# Autodesk Inventor assembly: ReleaseAssembly
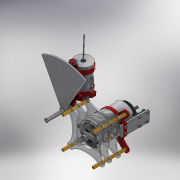
[picture p0: Inventor's stored thumbnail of the model, 180x180]
Saved by Autodesk Inventor 2018 (Build 220112000, 112)
## iProperties
Created: 2018-03-27
Part Number: ReleaseAssembly
Document SubType Name: Assembly
Designer: mansu
Author: mansu
## Documents named in this file (3)
- F:\OneDrive\Documents\2018 UBC\ELEC 391\Controller\cad\release\ReleaseAssembly.iam
- F:\OneDrive\Documents\2018 UBC\ELEC 391\Controller\cad\release\PitchAssembly.iam
- F:\OneDrive\Documents\2018 UBC\ELEC 391\Controller\cad\release\YawAssembly.iam
## Components (2 placed, 2 different names)
1. PitchAssembly:1 [sub-assembly] — Mate:2
2. YawAssembly:1 [sub-assembly] — Mate:1
## Relationships (2: Mate 2)
- Mate:1: YawAssembly:1
- Mate:2: PitchAssembly:1
